# Autodesk Inventor assembly: 車軸受け
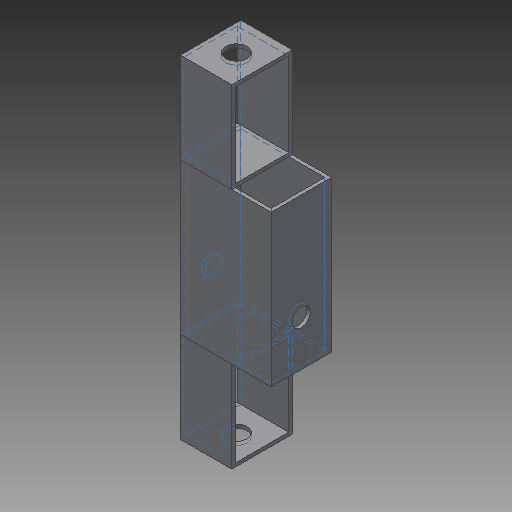
[picture p0: Inventor's stored thumbnail of the model, 512x512]
Saved by Autodesk Inventor 2018 (Build 220112000, 112)
## iProperties
Created: 2017-09-15
Part Number: 車軸受け
Material: 一般
Document SubType Name: Assembly
Designer: mura5
Author: mura5
## Documents named in this file (3)
- C:\Users\mura5\Documents\RBBR\cart\前足改\車軸受け改改\車軸受け.iam
- C:\Users\mura5\Documents\RBBR\cart\前足改\車軸受け改改\車軸受け1.ipt
- C:\Users\mura5\Documents\RBBR\cart\前足改\車軸受け改改\車軸受け2.ipt
## Components (3 placed, 2 different names)
1. 車軸受け1:1 — リジッド:1, リジッド:2
2. 車軸受け2:1 — リジッド:1
3. 車軸受け2:2 — リジッド:2
## Relationships (2: WeldJoint 2)
- リジッド:1 [WeldJoint]: 車軸受け1:1 ↔ 車軸受け2:1
- リジッド:2 [WeldJoint]: 車軸受け1:1 ↔ 車軸受け2:2
